# Autodesk Inventor assembly: flex_wheel_hub
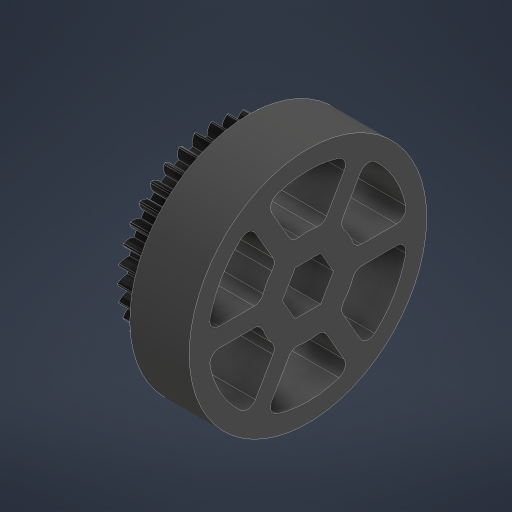
[picture p0: Inventor's stored thumbnail of the model, 512x512]
Saved by Autodesk Inventor 2024 (Build 280153000, 153)
## iProperties
Created: 2024-01-13
Part Number: flex_wheel_hub
Document SubType Name: Assembly
Designer: avere
Author: avere
## Documents named in this file (4)
- C:\Users\avere\Documents\rbp_cad\zoomba_v0.3\flex_wheel_hub.iam
- C:\Users\avere\Documents\rbp_cad\VEX-CAD-Inventor-1.41\Motion\Gears\LS 36T Gear.ipt
- C:\Users\avere\Documents\rbp_cad\VEX-CAD-Inventor-1.41\Motion\Wheels\Flex Wheels\2.000 Flex Wheel\2.000 60A .500.ipt
- C:\Users\avere\Documents\rbp_cad\VEX-CAD-Inventor-1.41\Motion\Wheels\Flex Wheels\2.000 Flex Wheel.ipt
## Components (2 placed, 2 different names)
1. LS 36T Gear:1 — Insert:1
2. 2.000 60A .500:1 — Insert:1
## Relationships (1: Insert 1)
- Insert:1: LS 36T Gear:1 ↔ 2.000 60A .500:1
